# Autodesk Inventor assembly: Extruder_Kit
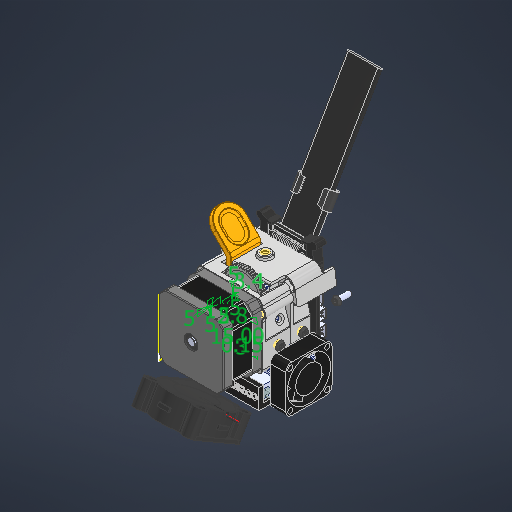
[picture p0: Inventor's stored thumbnail of the model, 512x512]
Saved by Autodesk Inventor 2027.1 (Build 311270010, 270A)
## iProperties
Created: 2026-09-19
Part Number: Extruder_Kit
Document SubType Name: Assembly
Designer: tdxt
Author: tdxt
## Documents named in this file (19)
- C:\Users\tdxt\OneDrive\Documents\GitHub\neptune3pro\Hardware\3D\Inventor\Extruder_Kit.iam
- C:\Users\tdxt\OneDrive\Documents\GitHub\neptune3pro\Hardware\3D\Inventor\Gearbox_Module(Ä¬ÈÏ-_flexible1).iam
- C:\Users\tdxt\OneDrive\Documents\GitHub\neptune3pro\Hardware\3D\Inventor\Nozzle_Module.iam
- C:\Users\tdxt\OneDrive\Documents\GitHub\neptune3pro\Hardware\3D\Inventor\Extruder PCBA.iam
- C:\Users\tdxt\OneDrive\Documents\GitHub\neptune3pro\Hardware\3D\Inventor\Extruder Shell_Kit.iam
- C:\Users\tdxt\OneDrive\Documents\GitHub\neptune3pro\Hardware\3D\Inventor\Level Sensor.ipt
- C:\Users\tdxt\OneDrive\Documents\GitHub\neptune3pro\Hardware\3D\Inventor\Hexagon Socket Button Head screw_M3x6.ipt
- C:\Users\tdxt\OneDrive\Documents\GitHub\neptune3pro\Hardware\3D\Inventor\Hexagon Socket Button Head screw_M3x30.ipt
- C:\Users\tdxt\OneDrive\Documents\GitHub\neptune3pro\Hardware\3D\Inventor\Hexagon Socket Button Head screw_M3x16.ipt
- C:\Users\tdxt\OneDrive\Documents\GitHub\neptune3pro\Hardware\3D\Inventor\Hexagon Socket Button Head screw_M3x8.ipt
- C:\Users\tdxt\OneDrive\Documents\GitHub\neptune3pro\Hardware\3D\Inventor\Hexagon Socket Countersunk Head screw_M3x35.ipt
- C:\Users\tdxt\OneDrive\Documents\GitHub\neptune3pro\Hardware\3D\Inventor\4015 Turbo Fan.ipt
- C:\Users\tdxt\OneDrive\Documents\GitHub\neptune3pro\Hardware\3D\Inventor\Cruciform Socket Button Head screw_PWM M2x10.ipt
- C:\Users\tdxt\OneDrive\Documents\GitHub\neptune3pro\Hardware\3D\Inventor\Fixing Plate_Extruder Fan(Ä¬ÈÏ).ipt
- C:\Users\tdxt\OneDrive\Documents\GitHub\neptune3pro\Hardware\3D\Inventor\Extruder Cable.ipt
- C:\Users\tdxt\OneDrive\Documents\GitHub\neptune3pro\Hardware\3D\Inventor\Fixing Plate_Extruder Cable(Ä¬ÈÏ).ipt
- C:\Users\tdxt\OneDrive\Documents\GitHub\neptune3pro\Hardware\3D\Inventor\Extruder Stepper Motor.iam
- C:\Users\tdxt\OneDrive\Documents\GitHub\neptune3pro\Hardware\3D\Misc Imports\3010 Axial Fan\3010 Axial Fan.ipt
- C:\Users\tdxt\OneDrive\Documents\GitHub\neptune3pro\Hardware\3D\Inventor\Bridge.ipt
## Components (32 placed, 18 different names)
1. Gearbox_Module(Ä¬ÈÏ-_flexible1) [sub-assembly] — Flush:2
2. Nozzle_Module [sub-assembly]
3. Extruder PCBA [sub-assembly]
4. Extruder Shell_Kit [sub-assembly]
5. Level Sensor — Flush:1
6. Hexagon Socket Button Head screw_M3x6
7. Hexagon Socket Button Head screw_M3x6:1
8. Hexagon Socket Button Head screw_M3x6:2
9. Hexagon Socket Button Head screw_M3x30
10. Hexagon Socket Button Head screw_M3x16
11. Hexagon Socket Button Head screw_M3x16:1
12. Hexagon Socket Button Head screw_M3x6:3
13. Hexagon Socket Button Head screw_M3x8
14. Hexagon Socket Button Head screw_M3x8:1
15. Hexagon Socket Button Head screw_M3x8:2
16. Hexagon Socket Countersunk Head screw_M3x35
17. Hexagon Socket Countersunk Head screw_M3x35:1
18. Hexagon Socket Countersunk Head screw_M3x35:2
19. 4015 Turbo Fan
20. Hexagon Socket Button Head screw_M3x6:4
21. Cruciform Socket Button Head screw_PWM M2x10
22. Cruciform Socket Button Head screw_PWM M2x10:1
23. Cruciform Socket Button Head screw_PWM M2x10:2
24. Fixing Plate_Extruder Fan(Ä¬ÈÏ)
25. Hexagon Socket Button Head screw_M3x16:2
26. Extruder Cable
27. Fixing Plate_Extruder Cable(Ä¬ÈÏ)
28. Hexagon Socket Button Head screw_M3x16:3
29. Extruder Stepper Motor:1 [sub-assembly]
30. 3010 Axial Fan:1
31. 3010 Axial Fan:2
32. Bridge:1 — Flush:1, Flush:2
## Relationships (2: Flush 2)
- Flush:1: Level Sensor ↔ Bridge:1
- Flush:2: Gearbox_Module(Ä¬ÈÏ-_flexible1) ↔ Bridge:1
